# Autodesk Inventor assembly: body
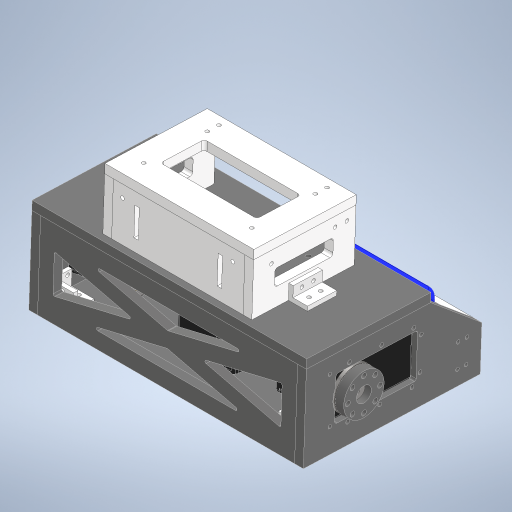
[picture p0: Inventor's stored thumbnail of the model, 512x512]
Saved by Autodesk Inventor 2024.3 (Build 283343000, 343)
## iProperties
Created: 2024-09-17
Part Number: body
Document SubType Name: Assembly
Designer: 구지현
Author: 구지현
## Documents named in this file (20)
- C:\Users\구지현\Desktop\19th_intern_kdy_robot\부품\Upper_Body\Body\body.iam
- C:\Users\구지현\Desktop\19th_intern_kdy_robot\부품\Upper_Body\Body\Back_Cover.ipt
- C:\Users\구지현\Desktop\19th_intern_kdy_robot\부품\Upper_Body\Body\body_fitting_parts.ipt
- C:\Users\구지현\Desktop\19th_intern_kdy_robot\부품\Upper_Body\Body\body_front.ipt
- C:\Users\구지현\Desktop\19th_intern_kdy_robot\부품\Upper_Body\Body\body_side.ipt
- C:\Users\구지현\Desktop\19th_intern_kdy_robot\부품\Upper_Body\Body\body_top.ipt
- C:\Users\구지현\Desktop\19th_intern_kdy_robot\부품\Upper_Body\Body\body_under.ipt
- C:\Users\구지현\Desktop\19th_intern_kdy_robot\부품\Upper_Body\Body\face_ front.ipt
- C:\Users\구지현\Desktop\19th_intern_kdy_robot\부품\Upper_Body\Body\face_ left.ipt
- C:\Users\구지현\Desktop\19th_intern_kdy_robot\부품\Upper_Body\Body\face_right.ipt
- C:\Users\구지현\Desktop\19th_intern_kdy_robot\부품\Upper_Body\Body\face_top.ipt
- C:\Users\구지현\Desktop\19th_intern_kdy_robot\부품\Upper_Body\Body\head fitting parts.ipt
- C:\Users\구지현\Desktop\19th_intern_kdy_robot\부품\Upper_Body\Body\head_fitting_parts_box.ipt
- C:\Users\구지현\Desktop\19th_intern_kdy_robot\부품\battery\Enrichpower_2200mAh_11.1V_30C.ipt
- C:\Users\구지현\Desktop\19th_intern_kdy_robot\부품\ROBOTIS(Inventor 2024 ver.)\다이나믹셀\MX-64T+idle.ipt.iam
- C:\Users\구지현\Desktop\19th_intern_kdy_robot\부품\ROBOTIS(Inventor 2024 ver.)\혼\64-106Horn.ipt
- C:\Users\구지현\Desktop\19th_intern_kdy_robot\부품\Upper_Body\Body\body_fitting_part_under.ipt
- C:\Users\구지현\Desktop\19th_intern_kdy_robot\부품\Upper_Body\Body\body_fitting_parts_right.ipt
- C:\Users\구지현\Desktop\19th_intern_kdy_robot\부품\Upper_Body\Body\hon_fitting_parts.ipt
- MX-64T+idle.ipt
## Components (30 placed, 19 different names)
1. Back_Cover:1 — 플러쉬:18, 메이트:14, 삽입:19, 삽입:20, 삽입:21, 삽입:22, 삽입:23, 삽입:24, 메이트:27, 메이트:28, 메이트:30, 메이트:32, 삽입:29, 삽입:30, 삽입:31, 삽입:32, 메이트:37
2. Body_Fitting_Parts:1 — 메이트:15, 메이트:16, 메이트:17, 삽입:26
3. Body_Front:1 — 플러쉬:12, 메이트:9, 메이트:10, 플러쉬:15, 메이트:12, 메이트:16, 메이트:19, 메이트:41, 메이트:42
4. Body_Side:1 — 플러쉬:13, 메이트:8, 플러쉬:14, 메이트:10, 플러쉬:17, 삽입:19, 삽입:20, 삽입:21, 삽입:22, 메이트:18, 삽입:25, 메이트:39, 삽입:36, 삽입:37
5. Body_Top:1 — 메이트:6, 삽입:1, 삽입:2, 삽입:5, 삽입:6, 삽입:14, 삽입:15, 플러쉬:12, 플러쉬:13, 메이트:8, 메이트:9, 플러쉬:14, 메이트:11, 플러쉬:16, 메이트:17, 메이트:20
6. Body_Under:1 — 메이트:12, 메이트:13, 플러쉬:17, 플러쉬:18, 메이트:14, 메이트:29, 메이트:31, 메이트:33, 메이트:40, 메이트:43, 삽입:40, 삽입:41
7. Face_ Front:1 — 플러쉬:6, 메이트:4, 플러쉬:7, 삽입:9, 플러쉬:10, 메이트:7, 삽입:18
8. Face_ Left:1 — 플러쉬:6, 메이트:4, 삽입:3, 삽입:4, 플러쉬:9, 삽입:10
9. Face_Right:1 — 메이트:6, 플러쉬:10, 메이트:7, 플러쉬:11, 삽입:11, 삽입:12, 삽입:13, 삽입:17
10. Face_Top:1 — 플러쉬:7, 플러쉬:9, 삽입:8, 플러쉬:11, 삽입:16
11. Head Fitting Parts:1 — 삽입:5, 삽입:6, 삽입:11, 삽입:12, 삽입:13, 삽입:14, 삽입:15
12. Head_Fitting_Parts_Box:1 — 삽입:8, 삽입:9, 삽입:10
13. Head_Fitting_Parts:2 — 삽입:1, 삽입:2, 삽입:3, 삽입:4
14. Head_Fitting_Parts_Box:2 — 삽입:16, 삽입:17, 삽입:18
15. Body_Side:2 — 플러쉬:15, 메이트:11, 플러쉬:16, 메이트:13, 삽입:23, 삽입:24, 메이트:15, 삽입:26, 메이트:38, 삽입:38, 삽입:39
16. Body_Fitting_Parts:2 — 메이트:18, 메이트:19, 메이트:20, 삽입:25
17. Body_Fitting_Parts:5 — 메이트:27, 메이트:28, 메이트:29, 삽입:32
18. Body_Fitting_Parts:6 — 메이트:30, 메이트:31, 메이트:32, 삽입:29, 삽입:30, 삽입:31
19. Enrichpower_2200mAh_11.1V_30C:1 — 메이트:33, 메이트:37
20. MX-64T+idle.ipt:1 [sub-assembly] — 삽입:35, 삽입:40, 삽입:41
21. MX-64T+idle.ipt:2 [sub-assembly] — 삽입:34, 삽입:38, 삽입:39
22. MX-64T+idle.ipt:3 [sub-assembly] — 삽입:33, 삽입:36, 삽입:37
23. 64-106Horn:1 — 삽입:35, 삽입:42
24. 64-106Horn:2 — 삽입:34, 삽입:44
25. 64-106Horn:3 — 삽입:33, 삽입:43
26. Body_Fitting_Parts_Under_Left:1 — 메이트:39, 메이트:40, 메이트:41
27. Body_Fitting_Parts_Right:1 — 메이트:38, 메이트:42, 메이트:43
28. Hon_Fitting_Parts:1 — 삽입:42
29. Hon_Fitting_Parts:2 — 삽입:43
30. Hon_Fitting_Parts:3 — 삽입:44
## Relationships (83: Insert 41, Mate 30, Flush 12)
- 플러쉬:6 [Flush]: Face_ Front:1 ↔ Face_ Left:1
- 메이트:4 [Mate]: Face_ Front:1 ↔ Face_ Left:1
- 메이트:6 [Mate]: Body_Top:1 ↔ Face_Right:1
- 삽입:1 [Insert]: Body_Top:1 ↔ Head_Fitting_Parts:2
- 삽입:2 [Insert]: Body_Top:1 ↔ Head_Fitting_Parts:2
- 삽입:3 [Insert]: Face_ Left:1 ↔ Head_Fitting_Parts:2
- 삽입:4 [Insert]: Face_ Left:1 ↔ Head_Fitting_Parts:2
- 삽입:5 [Insert]: Body_Top:1 ↔ Head Fitting Parts:1
- 삽입:6 [Insert]: Body_Top:1 ↔ Head Fitting Parts:1
- 플러쉬:7 [Flush]: Face_ Front:1 ↔ Face_Top:1
- 플러쉬:9 [Flush]: Face_ Left:1 ↔ Face_Top:1
- 삽입:8 [Insert]: Face_Top:1 ↔ Head_Fitting_Parts_Box:1
- 삽입:9 [Insert]: Face_ Front:1 ↔ Head_Fitting_Parts_Box:1
- 삽입:10 [Insert]: Face_ Left:1 ↔ Head_Fitting_Parts_Box:1
- 플러쉬:10 [Flush]: Face_ Front:1 ↔ Face_Right:1
- 메이트:7 [Mate]: Face_ Front:1 ↔ Face_Right:1
- 플러쉬:11 [Flush]: Face_Right:1 ↔ Face_Top:1
- 삽입:11 [Insert]: Face_Right:1 ↔ Head Fitting Parts:1
- 삽입:12 [Insert]: Face_Right:1 ↔ Head Fitting Parts:1
- 삽입:13 [Insert]: Face_Right:1 ↔ Head Fitting Parts:1
- 삽입:14 [Insert]: Body_Top:1 ↔ Head Fitting Parts:1
- 삽입:15 [Insert]: Body_Top:1 ↔ Head Fitting Parts:1
- 삽입:16 [Insert]: Face_Top:1 ↔ Head_Fitting_Parts_Box:2
- 삽입:17 [Insert]: Face_Right:1 ↔ Head_Fitting_Parts_Box:2
- 삽입:18 [Insert]: Face_ Front:1 ↔ Head_Fitting_Parts_Box:2
- 플러쉬:12 [Flush]: Body_Front:1 ↔ Body_Top:1
- 플러쉬:13 [Flush]: Body_Side:1 ↔ Body_Top:1
- 메이트:8 [Mate]: Body_Side:1 ↔ Body_Top:1
- 메이트:9 [Mate]: Body_Front:1 ↔ Body_Top:1
- 플러쉬:14 [Flush]: Body_Side:1 ↔ Body_Top:1
- 메이트:10 [Mate]: Body_Front:1 ↔ Body_Side:1
- 플러쉬:15 [Flush]: Body_Front:1 ↔ Body_Side:2
- 메이트:11 [Mate]: Body_Top:1 ↔ Body_Side:2
- 플러쉬:16 [Flush]: Body_Top:1 ↔ Body_Side:2
- 메이트:12 [Mate]: Body_Front:1 ↔ Body_Under:1
- 메이트:13 [Mate]: Body_Under:1 ↔ Body_Side:2
- 플러쉬:17 [Flush]: Body_Side:1 ↔ Body_Under:1
- 플러쉬:18 [Flush]: Back_Cover:1 ↔ Body_Under:1
- 메이트:14 [Mate]: Back_Cover:1 ↔ Body_Under:1
- 삽입:19 [Insert]: Back_Cover:1 ↔ Body_Side:1
- 삽입:20 [Insert]: Back_Cover:1 ↔ Body_Side:1
- 삽입:21 [Insert]: Back_Cover:1 ↔ Body_Side:1
- 삽입:22 [Insert]: Back_Cover:1 ↔ Body_Side:1
- 삽입:23 [Insert]: Back_Cover:1 ↔ Body_Side:2
- 삽입:24 [Insert]: Back_Cover:1 ↔ Body_Side:2
- 메이트:15 [Mate]: Body_Fitting_Parts:1 ↔ Body_Side:2
- 메이트:16 [Mate]: Body_Fitting_Parts:1 ↔ Body_Front:1
- 메이트:17 [Mate]: Body_Fitting_Parts:1 ↔ Body_Top:1
- 메이트:18 [Mate]: Body_Side:1 ↔ Body_Fitting_Parts:2
- 메이트:19 [Mate]: Body_Front:1 ↔ Body_Fitting_Parts:2
- 메이트:20 [Mate]: Body_Top:1 ↔ Body_Fitting_Parts:2
- 삽입:25 [Insert]: Body_Side:1 ↔ Body_Fitting_Parts:2
- 삽입:26 [Insert]: Body_Fitting_Parts:1 ↔ Body_Side:2
- 메이트:27 [Mate]: Back_Cover:1 ↔ Body_Fitting_Parts:5
- 메이트:28 [Mate]: Back_Cover:1 ↔ Body_Fitting_Parts:5
- 메이트:29 [Mate]: Body_Under:1 ↔ Body_Fitting_Parts:5
- 메이트:30 [Mate]: Back_Cover:1 ↔ Body_Fitting_Parts:6
- 메이트:31 [Mate]: Body_Under:1 ↔ Body_Fitting_Parts:6
- 메이트:32 [Mate]: Back_Cover:1 ↔ Body_Fitting_Parts:6
- 삽입:29 [Insert]: Back_Cover:1 ↔ Body_Fitting_Parts:6
- 삽입:30 [Insert]: Back_Cover:1 ↔ Body_Fitting_Parts:6
- 삽입:31 [Insert]: Back_Cover:1 ↔ Body_Fitting_Parts:6
- 삽입:32 [Insert]: Back_Cover:1 ↔ Body_Fitting_Parts:5
- 메이트:33 [Mate]: Body_Under:1 ↔ Enrichpower_2200mAh_11.1V_30C:1
- 삽입:33 [Insert]: MX-64T+idle.ipt:3 ↔ 64-106Horn:3
- 삽입:34 [Insert]: MX-64T+idle.ipt:2 ↔ 64-106Horn:2
- 삽입:35 [Insert]: MX-64T+idle.ipt:1 ↔ 64-106Horn:1
- 메이트:37 [Mate] (0.5 mm): Back_Cover:1 ↔ Enrichpower_2200mAh_11.1V_30C:1
- 메이트:38 [Mate]: Body_Side:2 ↔ Body_Fitting_Parts_Right:1
- 메이트:39 [Mate]: Body_Side:1 ↔ Body_Fitting_Parts_Under_Left:1
- 메이트:40 [Mate]: Body_Under:1 ↔ Body_Fitting_Parts_Under_Left:1
- 메이트:41 [Mate]: Body_Front:1 ↔ Body_Fitting_Parts_Under_Left:1
- 메이트:42 [Mate]: Body_Front:1 ↔ Body_Fitting_Parts_Right:1
- 메이트:43 [Mate]: Body_Under:1 ↔ Body_Fitting_Parts_Right:1
- 삽입:36 [Insert]: Body_Side:1 ↔ MX-64T+idle.ipt:3
- 삽입:37 [Insert]: Body_Side:1 ↔ MX-64T+idle.ipt:3
- 삽입:38 [Insert]: Body_Side:2 ↔ MX-64T+idle.ipt:2
- 삽입:39 [Insert]: Body_Side:2 ↔ MX-64T+idle.ipt:2
- 삽입:40 [Insert]: Body_Under:1 ↔ MX-64T+idle.ipt:1
- 삽입:41 [Insert]: Body_Under:1 ↔ MX-64T+idle.ipt:1
- 삽입:42 [Insert]: 64-106Horn:1 ↔ Hon_Fitting_Parts:1
- 삽입:43 [Insert]: 64-106Horn:3 ↔ Hon_Fitting_Parts:2
- 삽입:44 [Insert]: 64-106Horn:2 ↔ Hon_Fitting_Parts:3
